# Autodesk Inventor assembly: 211-04
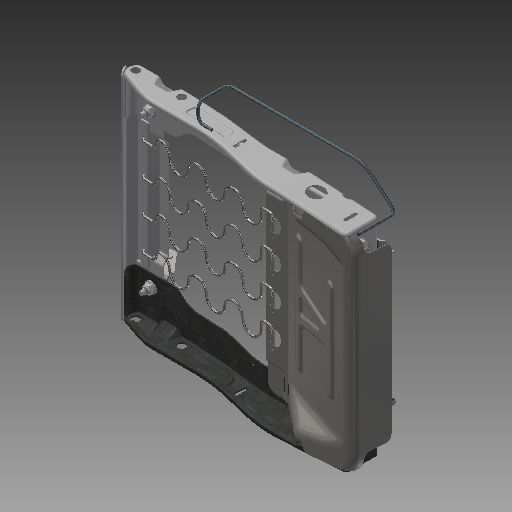
[picture p0: Inventor's stored thumbnail of the model, 512x512]
Saved by Autodesk Inventor 2019 (Build 230136000, 136)
## iProperties
Company: Autodesk Inc.
Created: 2007-12-25
Part Number: 211-04
Document SubType Name: Assembly
Designer: Autodesk Inc.
Mass: 4150.8 g
Surface Area: 6061.92 cm^2
Volume: 528.459 cm^3
Density: 7.85453 g/cm^3
Description: TOP FRAME ASSEMBLY
Component Category: Lower Component
Author: Inventor
## Documents named in this file (16)
- C:\TEMP\Car Seat\Workspace\Top Frame Assembly_MIR.iam
- C:\TEMP\Car Seat\Workspace\Top Back Plate.ipt
- C:\TEMP\Car Seat\Workspace\Top Frame Right Plate.ipt
- C:\TEMP\Car Seat\Workspace\Top Frame Left Plate.ipt
- C:\TEMP\Car Seat\Workspace\Front Top Shield.ipt
- C:\TEMP\Car Seat\Workspace\Corner Bracket R.ipt
- C:\TEMP\Car Seat\Workspace\Corner Bracket L.ipt
- C:\TEMP\Car Seat\Workspace\Bracket Spacer.ipt
- C:\TEMP\Car Seat\Workspace\Front Corner Bracket R.ipt
- C:\TEMP\Car Seat\Workspace\Front Corner Bracket L.ipt
- C:\TEMP\Car Seat\Workspace\Mounting Bracket Bolt.ipt
- C:\TEMP\Car Seat\Workspace\Mounting Bracket Nut.ipt
- C:\TEMP\Car Seat\Workspace\Spring Wire.ipt
- C:\TEMP\Car Seat\Workspace\Pivot Pin B.ipt
- C:\TEMP\Car Seat\Workspace\Bushing 3.ipt
- C:\TEMP\Car Seat\Workspace\Side Mounting Bar_MIR.ipt
## Components (29 placed, 15 different names)
1. Top Back Plate:1 — Flush:1, Flush:2, Mate:1, Insert:3, Insert:4, Mate:5, Angle:7
2. Top Frame Right Plate:1 — Angle:2, Mate:2, Mate:3, Insert:5, Insert:36, Insert:38
3. Top Frame Left Plate:1 — Angle:1, Insert:7, Insert:35, Insert:37
4. Front Top Shield:1 — Mate:2, Flush:3, Mate:3, Mate:4
5. Corner Bracket R:1 — Insert:3, Angle:4, Insert:13, Insert:33
6. Corner Bracket L:1 — Insert:4, Angle:3, Insert:14, Insert:34
7. Bracket Spacer:1 — Insert:5, Insert:6
8. Front Corner Bracket R:1 — Insert:6, Angle:5, Insert:9, Insert:29
9. Bracket Spacer:2 — Insert:7, Insert:8
10. Front Corner Bracket L:1 — Insert:8, Insert:10, Insert:30
11. Mounting Bracket Bolt:1 — Insert:9
12. Mounting Bracket Bolt:2 — Insert:10
13. Mounting Bracket Nut:2 — Insert:38
14. Mounting Bracket Nut:1 — Insert:37
15. Mounting Bracket Bolt:3 — Insert:13
16. Mounting Bracket Bolt:4 — Insert:14
17. Mounting Bracket Nut:4 — Insert:36
18. Mounting Bracket Nut:3 — Insert:35
19. Pivot Pin B:1 — Insert:29, Insert:31
20. Pivot Pin B:2 — Insert:30, Insert:32
21. Bushing 3:1 — Insert:31
22. Bushing 3:2 — Insert:32
23. Pivot Pin B:3 — Insert:33
24. Pivot Pin B:4 — Insert:34
25. Side Mounting Bar_MIR:1
26. Spring Wire:1 — Mate:4, Mate:5, Angle:7
27. Spring Wire:2
28. Spring Wire:3
29. Spring Wire:4
## Component patterns: (4 elements, first: Spring Wire:1)
## Relationships (37: Insert 22, Angle 7, Mate 5, Flush 3)
- Flush:1: Top Back Plate:1
- Flush:2: Top Back Plate:1
- Mate:1: Top Back Plate:1
- [Insert] (0.8 mm): Top Back Plate:1 ↔ Top Frame Right Plate:1
- [Insert] (0.8 mm): Top Back Plate:1 ↔ Top Frame Left Plate:1
- Angle:1 (0 deg): Top Frame Left Plate:1
- Angle:2 (180 deg): Top Frame Right Plate:1
- Mate:2: Top Frame Right Plate:1 ↔ Front Top Shield:1
- Flush:3: Front Top Shield:1
- Mate:3 (-76 mm): Top Frame Right Plate:1 ↔ Front Top Shield:1
- Insert:3: Top Back Plate:1 ↔ Corner Bracket R:1
- Insert:4: Top Back Plate:1 ↔ Corner Bracket L:1
- Angle:3 (180 deg): Corner Bracket L:1
- Angle:4 (0 deg): Corner Bracket R:1
- Insert:5: Top Frame Right Plate:1 ↔ Bracket Spacer:1
- Insert:6: Bracket Spacer:1 ↔ Front Corner Bracket R:1
- Angle:5 (0 deg): Front Corner Bracket R:1
- Insert:7: Top Frame Left Plate:1 ↔ Bracket Spacer:2
- Insert:8: Bracket Spacer:2 ↔ Front Corner Bracket L:1
- [Angle] (180 deg): Front Corner Bracket L:1
- Insert:9: Front Corner Bracket R:1 ↔ Mounting Bracket Bolt:1
- Insert:10: Front Corner Bracket L:1 ↔ Mounting Bracket Bolt:2
- Insert:13: Corner Bracket R:1 ↔ Mounting Bracket Bolt:3
- Insert:14: Corner Bracket L:1 ↔ Mounting Bracket Bolt:4
- Mate:4: Front Top Shield:1 ↔ Spring Wire:1
- Mate:5: Top Back Plate:1 ↔ Spring Wire:1
- Angle:7 (182.9 deg): Top Back Plate:1 ↔ Spring Wire:1
- Insert:29: Front Corner Bracket R:1 ↔ Pivot Pin B:1
- Insert:30: Front Corner Bracket L:1 ↔ Pivot Pin B:2
- Insert:31 (0.5 mm): Pivot Pin B:1 ↔ Bushing 3:1
- Insert:32 (0.5 mm): Pivot Pin B:2 ↔ Bushing 3:2
- Insert:33: Corner Bracket R:1 ↔ Pivot Pin B:3
- Insert:34: Corner Bracket L:1 ↔ Pivot Pin B:4
- Insert:35: Top Frame Left Plate:1 ↔ Mounting Bracket Nut:3
- Insert:36: Top Frame Right Plate:1 ↔ Mounting Bracket Nut:4
- Insert:37: Top Frame Left Plate:1 ↔ Mounting Bracket Nut:1
- Insert:38: Top Frame Right Plate:1 ↔ Mounting Bracket Nut:2
